# Autodesk Inventor assembly: FLUGGER FRT DOOR
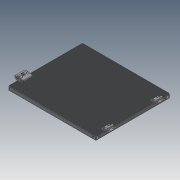
[picture p0: Inventor's stored thumbnail of the model, 180x180]
Saved by Autodesk Inventor 2020.3 (Build 243373000, 373)
## iProperties
RuleStatus: InUse
AfterDocSave0: file://Part Number Cleaner
Created: 2023-03-27
Catalog Web Link: https://www.janelia.org/
Vendor: HHMI: JRC - jET
Document SubType Name: Assembly
Designer: arnoldj
DESIGN DEPARTMENT: HHMI: JRC - jET
ALTERED ITEM PART NUMBER: N/A
ALTERED ITEM VENDOR: N/A
ALTERED ITEM DESCRIPTION: N/A
PART NUMBER - LEGACY: Standard
Author: arnoldj
Revision Number: 0
## Documents named in this file (7)
- C:\_WORKSPACE\DATA\PROJECTS\_PROJECTS BY LAB\CARD (LAB)\FLUGGER\FLUGGER FRT DOOR.iam
- C:\_WORKSPACE\DATA\PROJECTS\_PROJECTS BY LAB\CARD (LAB)\FLUGGER\FL_5537T36_524MML.ipt
- C:\_WORKSPACE\DATA\PROJECTS\_PROJECTS BY LAB\CARD (LAB)\FLUGGER\FL_5537T36_630MML.ipt
- C:\_WORKSPACE\DATA\COMMON\McMaster\MCMASTER 5537T863_30MM FRAMING CONN .ipt
- C:\_WORKSPACE\DATA\PROJECTS\_PROJECTS BY LAB\CARD (LAB)\FLUGGER\FLUGGER FRT DOOR PANEL.ipt
- C:\_WORKSPACE\DATA\COMMON\McMaster\MCMASTER 1467A109 HINGE.iam
- C:\_WORKSPACE\DATA\COMMON\McMaster\MCMASTER 5537T532_A.ipt
## Components (12 placed, 6 different names)
1. FL_5537T36_524MML:1 — Flush:1, Flush:3, Mate:6, Mate:10, Mate:20, Mate:25, Angle:1
2. FL_5537T36_524MML:2 — Mate:3, Flush:4, Mate:21, Mate:22, Mate:24
3. FL_5537T36_630MML:1 — Mate:4, Flush:5, Mate:11, Mate:12, Mate:14, Mate:23, Mate:26
4. FL_5537T36_630MML:2 — Mate:5, Flush:6, Mate:7, Mate:8, Mate:17, Mate:18
5. MCMASTER 5537T863_30MM FRAMING CONN :1 — Mate:10, Mate:11, Mate:12, Mate:25
6. MCMASTER 5537T863_30MM FRAMING CONN :2 — Mate:14, Mate:21, Mate:22, Mate:23
7. MCMASTER 5537T863_30MM FRAMING CONN :3 — Mate:17, Mate:18, Mate:24
8. MCMASTER 5537T863_30MM FRAMING CONN :4 — Mate:6, Mate:7, Mate:8, Mate:20
9. FLUGGER FRT DOOR PANEL:1 — Mate:26, Mate:27, Flush:7, Mate:28, Mate:29, Mate:30, Mate:31, Mate:32, Mate:33, Mate:34, Mate:35
10. MCMASTER 1467A109 HINGE:1 [sub-assembly] — Mate:28, Mate:29, Mate:30
11. MCMASTER 1467A109 HINGE:2 [sub-assembly] — Mate:31, Mate:32, Mate:33
12. MCMASTER 5537T532_A:1 — Mate:34, Mate:35, Angle:1
## Relationships (35: Mate 28, Flush 6, Angle 1)
- Flush:1: FL_5537T36_524MML:1
- Mate:3: FL_5537T36_524MML:2
- Flush:3: FL_5537T36_524MML:1
- Flush:4: FL_5537T36_524MML:2
- Mate:4: FL_5537T36_630MML:1
- Flush:5: FL_5537T36_630MML:1
- Mate:5: FL_5537T36_630MML:2
- Flush:6: FL_5537T36_630MML:2
- Mate:6: FL_5537T36_524MML:1 ↔ MCMASTER 5537T863_30MM FRAMING CONN :4
- Mate:7: FL_5537T36_630MML:2 ↔ MCMASTER 5537T863_30MM FRAMING CONN :4
- Mate:8: FL_5537T36_630MML:2 ↔ MCMASTER 5537T863_30MM FRAMING CONN :4
- Mate:10: FL_5537T36_524MML:1 ↔ MCMASTER 5537T863_30MM FRAMING CONN :1
- Mate:11: FL_5537T36_630MML:1 ↔ MCMASTER 5537T863_30MM FRAMING CONN :1
- Mate:12: FL_5537T36_630MML:1 ↔ MCMASTER 5537T863_30MM FRAMING CONN :1
- Mate:14: FL_5537T36_630MML:1 ↔ MCMASTER 5537T863_30MM FRAMING CONN :2
- Mate:17: FL_5537T36_630MML:2 ↔ MCMASTER 5537T863_30MM FRAMING CONN :3
- Mate:18: FL_5537T36_630MML:2 ↔ MCMASTER 5537T863_30MM FRAMING CONN :3
- Mate:20: FL_5537T36_524MML:1 ↔ MCMASTER 5537T863_30MM FRAMING CONN :4
- Mate:21: FL_5537T36_524MML:2 ↔ MCMASTER 5537T863_30MM FRAMING CONN :2
- Mate:22: FL_5537T36_524MML:2 ↔ MCMASTER 5537T863_30MM FRAMING CONN :2
- Mate:23: FL_5537T36_630MML:1 ↔ MCMASTER 5537T863_30MM FRAMING CONN :2
- Mate:24: FL_5537T36_524MML:2 ↔ MCMASTER 5537T863_30MM FRAMING CONN :3
- Mate:25: FL_5537T36_524MML:1 ↔ MCMASTER 5537T863_30MM FRAMING CONN :1
- Mate:26: FL_5537T36_630MML:1 ↔ FLUGGER FRT DOOR PANEL:1
- Mate:27: FLUGGER FRT DOOR PANEL:1
- Flush:7: FLUGGER FRT DOOR PANEL:1
- Mate:28: FLUGGER FRT DOOR PANEL:1 ↔ MCMASTER 1467A109 HINGE:1
- Mate:29: FLUGGER FRT DOOR PANEL:1 ↔ MCMASTER 1467A109 HINGE:1
- Mate:30: FLUGGER FRT DOOR PANEL:1 ↔ MCMASTER 1467A109 HINGE:1
- Mate:31: FLUGGER FRT DOOR PANEL:1 ↔ MCMASTER 1467A109 HINGE:2
- Mate:32: FLUGGER FRT DOOR PANEL:1 ↔ MCMASTER 1467A109 HINGE:2
- Mate:33: FLUGGER FRT DOOR PANEL:1 ↔ MCMASTER 1467A109 HINGE:2
- Mate:34: FLUGGER FRT DOOR PANEL:1 ↔ MCMASTER 5537T532_A:1
- Mate:35: FLUGGER FRT DOOR PANEL:1 ↔ MCMASTER 5537T532_A:1
- Angle:1 (0 deg): FL_5537T36_524MML:1 ↔ MCMASTER 5537T532_A:1
